# Autodesk Inventor assembly: Roller Shaft
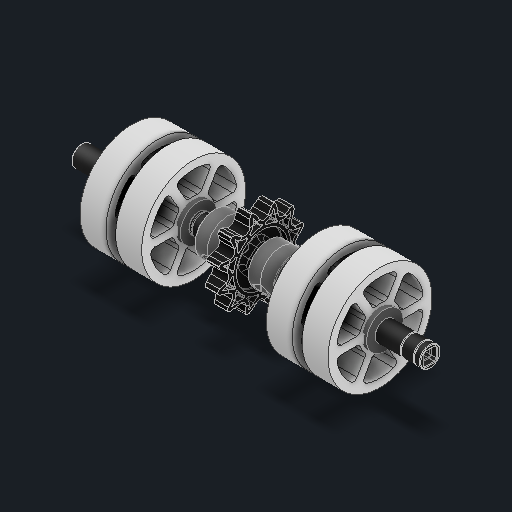
[picture p0: Inventor's stored thumbnail of the model, 512x512]
Saved by Autodesk Inventor 2025.1 (Build 291241000, 241)
## iProperties
Created: 2024-10-20
Part Number: Roller Shaft
Document SubType Name: Assembly
Designer: Averey Ku
Author: Averey Ku
## Documents named in this file (10)
- C:\Users\avere\VEX\High Stakes\CAD\V3\Intake\Conveyer\Roller Shaft.iam
- C:\Users\avere\VEX\High Stakes\CAD\ROBOPROS-CAD-Inventor\Motion\Sprockets\9P Sprocket\9P 12T Sprocket, No Insert.iam
- C:\Users\avere\VEX\High Stakes\CAD\ROBOPROS-CAD-Inventor\Motion\Shaft HS\HS Shaft Collar.ipt
- C:\Users\avere\VEX\High Stakes\CAD\ROBOPROS-CAD-Inventor\Motion\Shaft HS\HS Spacer\HSpacer .2500.ipt
- C:\Users\avere\VEX\High Stakes\CAD\ROBOPROS-CAD-Inventor\Motion\Shaft HS\HS Spacer\HSpacer .5000.ipt
- C:\Users\avere\VEX\High Stakes\CAD\ROBOPROS-CAD-Inventor\Motion\Shaft HS\HS Spacer\HSpacer .0625.ipt
- C:\Users\avere\VEX\High Stakes\CAD\ROBOPROS-CAD-Inventor\Motion\Shaft HS\HS Spacer\HSpacer .1250.ipt
- C:\Users\avere\VEX\High Stakes\CAD\ROBOPROS-CAD-Inventor\Motion\Sprockets\9P Sprocket.iam
- C:\Users\avere\VEX\High Stakes\CAD\ROBOPROS-CAD-Inventor\Motion\Shaft HS\HS Spacer.ipt
- C:\Users\avere\VEX\High Stakes\CAD\ROBOPROS-CAD-Inventor\Quick Assemblies\2.000 30A .500 With Adapters.iam
## Components (17 placed, 7 different names)
1. 9P 12T Sprocket, No Insert:1 [sub-assembly]
2. HS Shaft Collar:1 — Mate:2, Insert:34
3. HS Shaft Collar:2 — Insert:37
4. HSpacer .2500:10 — Insert:17, Insert:21
5. HSpacer .1250:11 — Insert:17
6. HSpacer .5000:12 — Insert:21, Insert:31
7. HSpacer .5000:13 — Insert:39
8. 2.000 30A .500 With Adapters:1 [sub-assembly] — Insert:25, Insert:41
9. 2.000 30A .500 With Adapters:2 [sub-assembly] — Insert:25, Insert:28
10. HSpacer .2500:14 — Insert:27, Insert:39
11. HSpacer .1250:15 — Insert:27, Insert:28
12. 2.000 30A .500 With Adapters:3 [sub-assembly] — Insert:31
13. 2.000 30A .500 With Adapters:4 [sub-assembly] — Insert:33
14. HSpacer .2500:16 — Insert:33
15. HSpacer .1250:17 — Insert:34
16. HSpacer .2500:18 — Insert:37, Insert:40
17. HSpacer .0625:19 — Insert:40, Insert:41
## Relationships (17: Insert 16, Mate 1)
- [Insert]: 9P 12T Sprocket, No Insert:1 ↔ HS Shaft Collar:1
- [Insert]: 9P 12T Sprocket, No Insert:1 ↔ HS Shaft Collar:2
- Mate:2 (6.35 mm): HS Shaft Collar:1
- Insert:17: HSpacer .2500:10 ↔ HSpacer .1250:11
- Insert:21: HSpacer .2500:10 ↔ HSpacer .5000:12
- Insert:25: 2.000 30A .500 With Adapters:1 ↔ 2.000 30A .500 With Adapters:2
- Insert:27: HSpacer .2500:14 ↔ HSpacer .1250:15
- Insert:28: 2.000 30A .500 With Adapters:2 ↔ HSpacer .1250:15
- [Insert]: 2.000 30A .500 With Adapters:3 ↔ 2.000 30A .500 With Adapters:4
- Insert:31: HSpacer .5000:12 ↔ 2.000 30A .500 With Adapters:3
- [Insert]: HSpacer .2500:16 ↔ HSpacer .1250:17
- Insert:33: 2.000 30A .500 With Adapters:4 ↔ HSpacer .2500:16
- Insert:34: HS Shaft Collar:1 ↔ HSpacer .1250:17
- Insert:37: HS Shaft Collar:2 ↔ HSpacer .2500:18
- Insert:39: HSpacer .5000:13 ↔ HSpacer .2500:14
- Insert:40: HSpacer .2500:18 ↔ HSpacer .0625:19
- Insert:41: 2.000 30A .500 With Adapters:1 ↔ HSpacer .0625:19
## Named parameters: d35_d30 = 0 mm, d37_d21 = 0 mm
